# Autodesk Inventor assembly: placa sensor de mangal
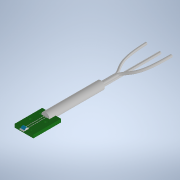
[picture p0: Inventor's stored thumbnail of the model, 180x180]
Saved by Autodesk Inventor 2021 (Build 250183000, 183)
## iProperties
Company: A Company
Created: 2021-05-08
Part Number: placa sensor de mangal
Description: KiCad electronic assembly
Document SubType Name: Assembly
Designer: Willy.exe
Authority: Unknown
Sending System: KiCad to STEP converter
Preprocessor: Open CASCADE STEP processor 6.9
Title: placa sensor de mangal.step
Author: An Author
## Documents named in this file (4)
- D:\GitHub\Sensor de mangal\PCBsensorMangal\placa sensor de mangal.iam
- D:\GitHub\Sensor de mangal\PCBsensorMangal\COMPOUND.ipt
- D:\Disenos Inventor\Sensor de mancal\Sensor pt100.ipt
- D:\Disenos Inventor\Sensor de mancal\Cable sensor.ipt
## Components (3 placed, 3 different names)
1. 7 — Rígido:1, Rígido:2
2. Sensor pt100:1 — Rígido:1
3. Cable sensor:1 — Rígido:2
## Relationships (2: WeldJoint 2)
- Rígido:1 [WeldJoint]: 7 ↔ Sensor pt100:1
- Rígido:2 [WeldJoint] (-3 mm): 7 ↔ Cable sensor:1
